# Autodesk Inventor assembly: oska-assembly
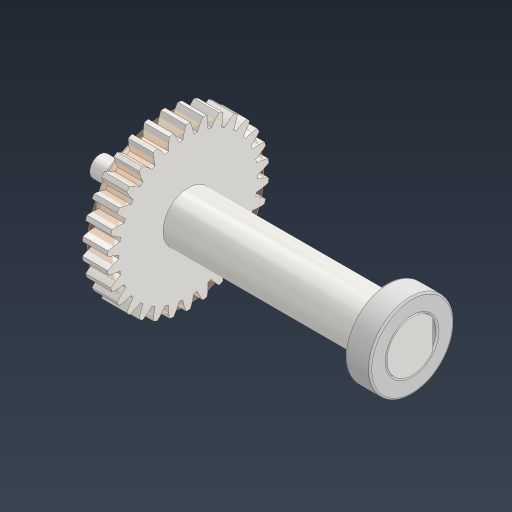
[picture p0: Inventor's stored thumbnail of the model, 512x512]
Saved by Autodesk Inventor 2023 (Build 270158000, 158)
## iProperties
Created: 2026-03-09
Part Number: oska-assembly
Document SubType Name: Assembly
Designer: szymo
Author: szymo
## Documents named in this file (4)
- D:\tech\robotyka\robots\evangelion-turbo\inventor-project\oska-assembly.iam
- D:\tech\robotyka\robots\evangelion-turbo\inventor-project\shaft.ipt
- D:\tech\robotyka\robots\evangelion-turbo\inventor-project\BigGear.iam
- D:\tech\robotyka\robots\evangelion-turbo\inventor-project\ball-bearing.ipt
## Components (4 placed, 3 different names)
1. Shaft:1 — Mate:1, Mate:2, Mate:3, Mate:4, Mate:6
2. Spur Gears:1 [sub-assembly] — Mate:1, Mate:2, Mate:5
3. ball-bearing:1 — Mate:4, Mate:6
4. ball-bearing:2 — Mate:3, Mate:5
## Relationships (6: Mate 6)
- Mate:1: Shaft:1 ↔ Spur Gears:1
- Mate:2: Shaft:1 ↔ Spur Gears:1
- Mate:3: Shaft:1 ↔ ball-bearing:2
- Mate:4: Shaft:1 ↔ ball-bearing:1
- Mate:5 (0.1 mm): Spur Gears:1 ↔ ball-bearing:2
- Mate:6: Shaft:1 ↔ ball-bearing:1
